# Autodesk Inventor assembly: Ramp - Side - Trapezoid Assembly_MIR2
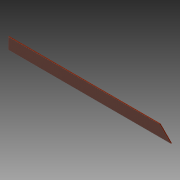
[picture p0: Inventor's stored thumbnail of the model, 180x180]
Saved by Autodesk Inventor 2015 (Build 190159000, 159)
## iProperties
Created: 2015-01-20
Part Number: Ramp - Side - Trapezoid Assembly_MIR2
Document SubType Name: Assembly
Designer: peters
Author: Peter
## Documents named in this file (3)
- C:\Users\peters\Documents\FIRST-Team-1719-CAD-Team\2015 Playing Field\Team 1719 Practice Field\Scoring Platform Version 2 - Construction Design\Ramp - Side - Trapezoid Assembly_MIR2.iam
- C:\Users\peters\Documents\FIRST-Team-1719-CAD-Team\2015 Playing Field\Team 1719 Practice Field\Scoring Platform Version 2 - Construction Design\Ramp - Side - Trapezoid Polycarbonate 125_MIR2.ipt
- C:\Users\peters\Documents\FIRST-Team-1719-CAD-Team\2015 Playing Field\Team 1719 Practice Field\Scoring Platform Version 2 - Construction Design\Ramp - Side - Trapezoid Plywood 375_MIR2.ipt
## Components (2 placed, 2 different names)
1. Ramp - Side - Trapezoid Polycarbonate 125_MIR2:1 — Mate:1, Flush:2, Flush:1
2. Ramp - Side - Trapezoid Plywood 375_MIR2:1 — Mate:1, Flush:2, Flush:1
## Relationships (3: Flush 2, Mate 1)
- Mate:1: Ramp - Side - Trapezoid Polycarbonate 125_MIR2:1 ↔ Ramp - Side - Trapezoid Plywood 375_MIR2:1
- Flush:2: Ramp - Side - Trapezoid Polycarbonate 125_MIR2:1 ↔ Ramp - Side - Trapezoid Plywood 375_MIR2:1
- Flush:1: Ramp - Side - Trapezoid Polycarbonate 125_MIR2:1 ↔ Ramp - Side - Trapezoid Plywood 375_MIR2:1
